# Autodesk Inventor assembly: Frame
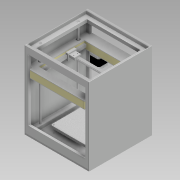
[picture p0: Inventor's stored thumbnail of the model, 180x180]
Saved by Autodesk Inventor 2016 (Build 200138000, 138)
## iProperties
Created: 2017-05-15
Part Number: Frame
Document SubType Name: Assembly
Designer: 31745
Author: 31745
## Documents named in this file (14)
- H:\Projects\Printer #2\Printer2\IAM\Frame.iam
- H:\Projects\Printer #2\Printer2\IPT\Machined Parts\Base.ipt
- H:\Projects\Printer #2\Printer2\IPT\Machined Parts\Print Bed.ipt
- H:\Projects\Printer #2\Printer2\IPT\Machined Parts\Smooth Rod Brace Bottom.ipt
- H:\Projects\Printer #2\Printer2\IPT\Purchased Parts\8mm smooth rod.ipt
- H:\Projects\Printer #2\Printer2\IPT\Machined Parts\Carriage Sheet.ipt
- H:\Projects\Printer #2\Printer2\IPT\Machined Parts\Left Face.ipt
- H:\Projects\Printer #2\Printer2\IPT\Machined Parts\Carriage Filler.ipt
- H:\Projects\Printer #2\Printer2\IPT\Purchased Parts\lm8uu rough model.ipt
- H:\Projects\Printer #2\Printer2\IPT\Machined Parts\Front Face.ipt
- H:\Projects\Printer #2\Printer2\IPT\Machined Parts\Top Sheet.ipt
- H:\Projects\Printer #2\Printer2\IPT\Purchased Parts\MGN12.ipt
- H:\Projects\Printer #2\Printer2\IPT\Purchased Parts\MGN Block.ipt
- H:\Projects\Printer #2\Printer2\IPT\Purchased Parts\M1173041- NEMA 17.ipt
## Components (29 placed, 13 different names)
1. Base:1 — Mate:1, Mate:2, Mate:3, Mate:4, Flush:3, Mate:9, Mate:10, Mate:11, Mate:12, Mate:20, Flush:15, Mate:21, Flush:16, Flush:17
2. Print Bed:1 — Mate:1, Mate:2, Mate:3
3. Smooth Rod Brace Bottom:1 — Mate:4, Flush:3, Mate:5, Mate:6, Mate:7, Mate:8, Mate:18, Mate:19, Flush:23, Mate:44
4. 8mm smooth rod:1 — Mate:8, Mate:11, Mate:23, Mate:29
5. 8mm smooth rod:2 — Mate:5, Mate:9, Mate:24, Mate:28
6. 8mm smooth rod:3 — Mate:7, Mate:10, Mate:22
7. 8mm smooth rod:4 — Mate:6, Mate:12, Mate:25
8. Carriage Sheet:1 — Flush:5, Flush:6, Mate:17, Mate:45, Mate:46
9. Carriage Sheet:2 — Flush:5, Flush:6, Mate:16, Flush:13, Flush:14, Flush:23, Flush:25, Flush:28, Flush:34
10. Carriage Filler:1 — Mate:16, Mate:17, Flush:13, Flush:14, Flush:24, Mate:33, Mate:34, Mate:35, Mate:36, Flush:40
11. Left Face:1 — Mate:18, Flush:15, Mate:21, Flush:16, Flush:24, Mate:27, Flush:31, Mate:31
12. Left Face:2 — Mate:19, Mate:20, Flush:17, Mate:26, Flush:29, Flush:30, Flush:32, Flush:33
13. lm8uu rough model:1 — Mate:23, Flush:27, Flush:28
14. lm8uu rough model:2 — Flush:25, Mate:22
15. lm8uu rough model:3 — Mate:24, Flush:26
16. lm8uu rough model:4 — Mate:25, Flush:26, Flush:27
17. Front Face:1 — Mate:27, Flush:31, Flush:32, Mate:32
18. Front Face:2 — Mate:26, Flush:29, Flush:30
19. Smooth Rod Brace Bottom:2 — Mate:28, Mate:29, Flush:33, Mate:30
20. Top Sheet:1 — Mate:30, Mate:31, Mate:32
21. MGN12:1 — Flush:34, Mate:33, Mate:34, Flush:35, Mate:37, Mate:40
22. MGN12:2 — Mate:35, Flush:35, Mate:36, Mate:38, Mate:39
23. MGN Block:1 — Mate:37, Mate:40, Flush:36, Mate:43, Flush:37, Flush:38
24. MGN Block:2 — Mate:38, Mate:39, Flush:36
25. MGN12:3 — Mate:43, Flush:37, Flush:38
26. MGN Block:3
27. M1173041- NEMA 17:1 — Mate:44
28. M1173041- NEMA 17:2 — Mate:46, Flush:39, Flush:40
29. M1173041- NEMA 17:3 — Mate:45, Flush:39
## Relationships (69: Mate 43, Flush 26)
- Mate:1: Base:1 ↔ Print Bed:1
- Mate:2: Base:1 ↔ Print Bed:1
- Mate:3 (19.05 mm): Base:1 ↔ Print Bed:1
- Mate:4: Base:1 ↔ Smooth Rod Brace Bottom:1
- Flush:3: Base:1 ↔ Smooth Rod Brace Bottom:1
- Mate:5: Smooth Rod Brace Bottom:1 ↔ 8mm smooth rod:2
- Mate:6: Smooth Rod Brace Bottom:1 ↔ 8mm smooth rod:4
- Mate:7: Smooth Rod Brace Bottom:1 ↔ 8mm smooth rod:3
- Mate:8: Smooth Rod Brace Bottom:1 ↔ 8mm smooth rod:1
- Mate:9: Base:1 ↔ 8mm smooth rod:2
- Mate:10: Base:1 ↔ 8mm smooth rod:3
- Mate:11: Base:1 ↔ 8mm smooth rod:1
- Mate:12: Base:1 ↔ 8mm smooth rod:4
- Flush:5: Carriage Sheet:1 ↔ Carriage Sheet:2
- Flush:6: Carriage Sheet:1 ↔ Carriage Sheet:2
- Mate:16: Carriage Sheet:2 ↔ Carriage Filler:1
- Mate:17: Carriage Sheet:1 ↔ Carriage Filler:1
- Flush:13: Carriage Sheet:2 ↔ Carriage Filler:1
- Flush:14: Carriage Sheet:2 ↔ Carriage Filler:1
- Mate:18: Smooth Rod Brace Bottom:1 ↔ Left Face:1
- Mate:19: Smooth Rod Brace Bottom:1 ↔ Left Face:2
- Mate:20: Base:1 ↔ Left Face:2
- Flush:15: Base:1 ↔ Left Face:1
- Mate:21: Base:1 ↔ Left Face:1
- Flush:16: Base:1 ↔ Left Face:1
- Flush:17: Base:1 ↔ Left Face:2
- Flush:23: Smooth Rod Brace Bottom:1 ↔ Carriage Sheet:2
- Flush:24: Carriage Filler:1 ↔ Left Face:1
- Flush:25: Carriage Sheet:2 ↔ lm8uu rough model:2
- Mate:22: 8mm smooth rod:3 ↔ lm8uu rough model:2
- Mate:23: 8mm smooth rod:1 ↔ lm8uu rough model:1
- Mate:24: 8mm smooth rod:2 ↔ lm8uu rough model:3
- Mate:25: 8mm smooth rod:4 ↔ lm8uu rough model:4
- Flush:26: lm8uu rough model:3 ↔ lm8uu rough model:4
- Flush:27: lm8uu rough model:1 ↔ lm8uu rough model:4
- Flush:28: Carriage Sheet:2 ↔ lm8uu rough model:1
- Mate:26: Left Face:2 ↔ Front Face:2
- Flush:29: Left Face:2 ↔ Front Face:2
- Flush:30: Left Face:2 ↔ Front Face:2
- Mate:27: Left Face:1 ↔ Front Face:1
- Flush:31: Left Face:1 ↔ Front Face:1
- Flush:32: Left Face:2 ↔ Front Face:1
- Mate:28: 8mm smooth rod:2 ↔ Smooth Rod Brace Bottom:2
- Mate:29: 8mm smooth rod:1 ↔ Smooth Rod Brace Bottom:2
- Flush:33: Left Face:2 ↔ Smooth Rod Brace Bottom:2
- Mate:30: Smooth Rod Brace Bottom:2 ↔ Top Sheet:1
- Mate:31: Left Face:1 ↔ Top Sheet:1
- Mate:32: Front Face:1 ↔ Top Sheet:1
- Flush:34 (8.9916 mm): Carriage Sheet:2 ↔ MGN12:1
- Mate:33: Carriage Filler:1 ↔ MGN12:1
- Mate:34: Carriage Filler:1 ↔ MGN12:1
- Mate:35: Carriage Filler:1 ↔ MGN12:2
- Flush:35: MGN12:1 ↔ MGN12:2
- Mate:36: Carriage Filler:1 ↔ MGN12:2
- Mate:37: MGN12:1 ↔ MGN Block:1
- Mate:38: MGN12:2 ↔ MGN Block:2
- Mate:39: MGN12:2 ↔ MGN Block:2
- Mate:40: MGN12:1 ↔ MGN Block:1
- Flush:36: MGN Block:1 ↔ MGN Block:2
- [Mate]: MGN12:3 ↔ MGN Block:3
- [Mate]: MGN12:3 ↔ MGN Block:3
- Mate:43: MGN Block:1 ↔ MGN12:3
- Flush:37 (9.4488 mm): MGN Block:1 ↔ MGN12:3
- Flush:38 (11.3538 mm): MGN Block:1 ↔ MGN12:3
- Mate:44: Smooth Rod Brace Bottom:1 ↔ M1173041- NEMA 17:1
- Mate:45: Carriage Sheet:1 ↔ M1173041- NEMA 17:3
- Mate:46: Carriage Sheet:1 ↔ M1173041- NEMA 17:2
- Flush:39: M1173041- NEMA 17:2 ↔ M1173041- NEMA 17:3
- Flush:40: Carriage Filler:1 ↔ M1173041- NEMA 17:2
## Named parameters: d76_d71 = 0 mm, d77_d74 = 0 mm
